# Autodesk Inventor assembly: Marcos
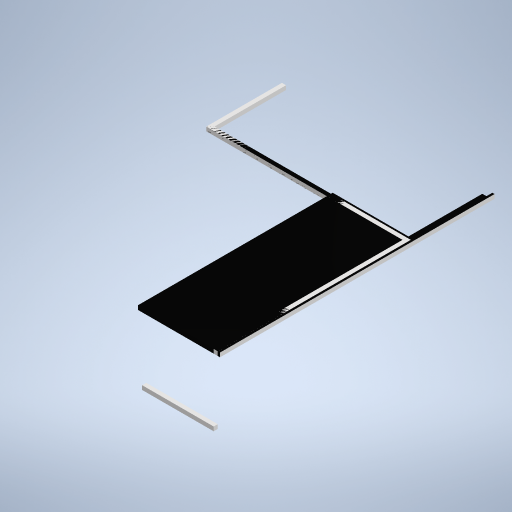
[picture p0: Inventor's stored thumbnail of the model, 512x512]
Saved by Autodesk Inventor 2024 (Build 280153000, 153)
## iProperties
Created: 2023-07-05
Part Number: Marcos
Document SubType Name: Assembly
Designer: sergi
Author: sergi
## Documents named in this file (6)
- C:\Users\sergi\OneDrive\Escritorio\Piso\Escritorio Piso\Marcos.iam
- C:\Users\sergi\OneDrive\Escritorio\Piso\Escritorio Piso\Barra1.ipt
- C:\Users\sergi\OneDrive\Escritorio\Piso\Escritorio Piso\BarraMarco1.1.ipt
- C:\Users\sergi\OneDrive\Escritorio\Piso\Escritorio Piso\BarraMarco1.2.ipt
- C:\Users\sergi\OneDrive\Escritorio\Piso\Escritorio Piso\BarraMarco2.1.ipt
- C:\Users\sergi\OneDrive\Escritorio\Piso\Escritorio Piso\BarraMarco2.2.ipt
## Components (5 placed, 5 different names)
1. Barra1:1 — Nivelación:1, Nivelación:2, Nivelación:3, Nivelación:4
2. BarraMarco1.1:1
3. BarraMarco1.2:1 — Nivelación:1, Nivelación:2
4. BarraMarco2.1:1 — Nivelación:3
5. BarraMarco2.2:1 — Nivelación:4
## Relationships (4: Flush 4)
- Nivelación:1 [Flush]: Barra1:1 ↔ BarraMarco1.2:1
- Nivelación:2 [Flush]: Barra1:1 ↔ BarraMarco1.2:1
- Nivelación:3 [Flush]: Barra1:1 ↔ BarraMarco2.1:1
- Nivelación:4 [Flush]: Barra1:1 ↔ BarraMarco2.2:1
